# Autodesk Inventor assembly: Top Crossbrace
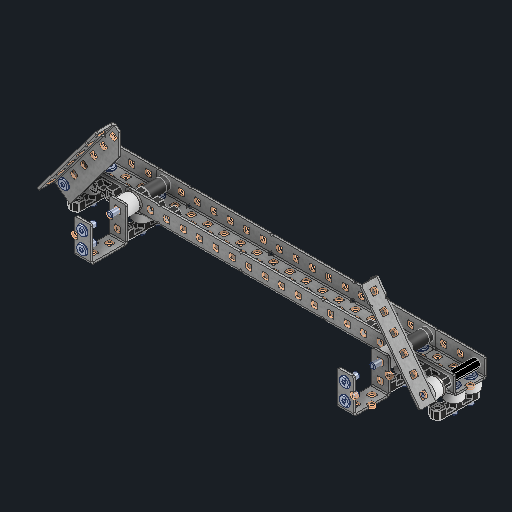
[picture p0: Inventor's stored thumbnail of the model, 512x512]
Saved by Autodesk Inventor 2025 (Build 290162000, 162)
## iProperties
Created: 2024-10-20
Part Number: Top Crossbrace
Document SubType Name: Assembly
Designer: Averey Ku
Author: Averey Ku
## Documents named in this file (26)
- D:\VEX\High Stakes\CAD\V2\Chassis\Structure\Top Crossbrace.iam
- D:\VEX\High Stakes\CAD\ROBOPROS-CAD-Inventor\Structure\C Channel\Aluminum 1x2x1\Alu C 1x2x1x17.ipt
- D:\VEX\High Stakes\CAD\ROBOPROS-CAD-Inventor\Structure\C Channel\Aluminum 2x2x2\Alu C 2x2x2x1.ipt
- D:\VEX\High Stakes\CAD\ROBOPROS-CAD-Inventor\Motion\Spacers\Spacer Nylon .500 OD\NSpacer White .500 OD x .375.ipt
- D:\VEX\High Stakes\CAD\ROBOPROS-CAD-Inventor\Motion\Spacers\Spacer Nylon .500 OD.ipt
- D:\VEX\High Stakes\CAD\ROBOPROS-CAD-Inventor\Motion\Spacers\Washer Steel\SWasher .500 OD x .062500.ipt
- D:\VEX\High Stakes\CAD\ROBOPROS-CAD-Inventor\Motion\Shaft LS\Bearing Flat Low Profile.ipt
- D:\VEX\High Stakes\CAD\ROBOPROS-CAD-Inventor\Motion\Spacers\Washer Steel\SWasher .500 OD x .062500\SWasher .500 OD x .062500.ipt
- D:\VEX\High Stakes\CAD\ROBOPROS-CAD-Inventor\Motion\Spacers\Spacer Nylon .375 OD\NSpacer .375 OD x .125.ipt
- D:\VEX\High Stakes\CAD\ROBOPROS-CAD-Inventor\Motion\Spacers\Spacer Nylon .375 OD.ipt
- D:\VEX\High Stakes\CAD\ROBOPROS-CAD-Inventor\Motion\Spacers\Spacer Nylon .375 OD\NSpacer .375 OD x .500.ipt
- D:\VEX\High Stakes\CAD\ROBOPROS-CAD-Inventor\Structure\Hardware\Screw Steel - Star\SScrew Star Smooth 1.750.ipt
- D:\VEX\High Stakes\CAD\ROBOPROS-CAD-Inventor\Structure\Hardware\Screw Steel - Star.ipt
- D:\VEX\High Stakes\CAD\ROBOPROS-CAD-Inventor\Structure\Hardware\Screw Shoulder Robosource\SScrew Shoulder Smooth .375 x .12.ipt
- D:\VEX\High Stakes\CAD\ROBOPROS-CAD-Inventor\Structure\Hardware\Screw Shoulder Robosource.ipt
- D:\VEX\High Stakes\CAD\ROBOPROS-CAD-Inventor\Motion\Spacers\Spacer Nylon .500 OD\NSpacer White .500 OD x .250.ipt
- D:\VEX\High Stakes\CAD\ROBOPROS-CAD-Inventor\Structure\Hardware\Screw Steel - Star\SScrew Star Smooth .750.ipt
- D:\VEX\High Stakes\CAD\ROBOPROS-CAD-Inventor\Structure\C Channel\Aluminum 1x2x1\Alu C 1x2x1x23.ipt
- D:\VEX\High Stakes\CAD\ROBOPROS-CAD-Inventor\Structure\Standoff\Standoff .875.ipt
- D:\VEX\High Stakes\CAD\ROBOPROS-CAD-Inventor\Structure\Standoff.ipt
- D:\VEX\High Stakes\CAD\ROBOPROS-CAD-Inventor\Structure\C Channel\Aluminum 1x3x1 Half Thick Cut\Alu C Half Thick 1x3x1x6.ipt
- D:\VEX\High Stakes\CAD\ROBOPROS-CAD-Inventor\Structure\Hardware\Screw Steel - Star\SScrew Star Smooth .875.ipt
- D:\VEX\High Stakes\CAD\ROBOPROS-CAD-Inventor\Structure\Hardware\Screw Steel - Star\SScrew Star Smooth .290.ipt
- D:\VEX\High Stakes\CAD\V2\Chassis\Structure\Right\Alu C 2x2x2x1 Right.ipt
- D:\VEX\High Stakes\CAD\V2\Chassis\Structure\Right\Bearing Flat Low Profile Right.ipt
- D:\VEX\High Stakes\CAD\V2\Chassis\Structure\Right\Alu C Half Thick 1x3x1x6 Right.ipt
## Components (54 placed, 19 different names)
1. Alu C 1x2x1x23:1 — Insert:23, Flush:2, Insert:28, Insert:29, Insert:30, Insert:32, Insert:33, Insert:34, Mate:6, Insert:39, Insert:40, Insert:51
2. Alu C 1x2x1x17:1 — Insert:3, Insert:5, Mate:2, Insert:15, Flush:1, Flush:2
3. SScrew Shoulder Smooth .375 x .12:3 — Insert:52
4. Alu C 2x2x2x1:1 — Insert:2, Insert:16, Insert:52
5. NSpacer White .500 OD x .375:1 — Insert:2, Insert:4
6. Bearing Flat Low Profile:1 — Insert:3, Mate:2, Insert:12
7. SWasher .500 OD x .062500:1 — Insert:4, Insert:5, Insert:23
8. NSpacer .375 OD x .125:1 — Insert:11
9. NSpacer .375 OD x .500:2 — Insert:11, Insert:12
10. SScrew Star Smooth 1.750:1 — Insert:15
11. SScrew Shoulder Smooth .375 x .12:1 — Insert:16
12. Alu C Half Thick 1x3x1x6:1 — Insert:33, Insert:36, Insert:38
13. Bearing Flat Low Profile:8 — Insert:34, Mate:6, Insert:37
14. NSpacer White .500 OD x .250:14 — Insert:36
15. SWasher .500 OD x .062500:3 — Insert:37
16. SScrew Star Smooth .875:14 — Insert:38
17. Standoff .875:1 — Insert:39
18. SScrew Star Smooth .290:15 — Insert:40
19. SScrew Shoulder Smooth .375 x .12:4 — Insert:53
20. Alu C 2x2x2x1 Right:1 — Insert:41, Insert:45, Insert:53
21. NSpacer White .500 OD x .375:15 — Insert:41, Insert:42
22. Bearing Flat Low Profile Right:1 — Insert:43
23. SWasher .500 OD x .062500:4 — Insert:42
24. NSpacer .375 OD x .125:3 — Insert:44
25. NSpacer .375 OD x .500:4 — Insert:43, Insert:44
26. SScrew Star Smooth 1.750:16
27. SScrew Shoulder Smooth .375 x .12:2 — Insert:45
28. Alu C Half Thick 1x3x1x6 Right:1 — Insert:48, Insert:50
29. Bearing Flat Low Profile Right:3 — Insert:49
30. NSpacer White .500 OD x .250:18 — Insert:48
31. SWasher .500 OD x .062500:5 — Insert:49
32. SScrew Star Smooth .875:19 — Insert:50
33. Standoff .875:2
34. SScrew Star Smooth .290:20
35. NSpacer White .500 OD x .250:7 — Insert:32
36. NSpacer White .500 OD x .250:6 — Insert:30, Insert:31
37. Bearing Flat Low Profile:4 — Insert:31
38. SScrew Star Smooth .750:7 — Insert:29
39. SScrew Star Smooth .750:6 — Insert:28
40. NSpacer White .500 OD x .250:8
41. NSpacer White .500 OD x .250:9
42. Bearing Flat Low Profile:5
43. SScrew Star Smooth .750:8
44. SScrew Star Smooth .750:9
45. NSpacer White .500 OD x .250:16 — Insert:47, Insert:51
46. NSpacer White .500 OD x .250:17 — Insert:46, Mate:7
47. Bearing Flat Low Profile Right:2 — Insert:46, Insert:47
48. SScrew Star Smooth .750:17
49. SScrew Star Smooth .750:18 — Mate:7
50. NSpacer White .500 OD x .250:19
51. NSpacer White .500 OD x .250:20
52. Bearing Flat Low Profile Right:4
53. SScrew Star Smooth .750:21
54. SScrew Star Smooth .750:22
## Component patterns: Drivebay Attachments Left (2 elements), Drivebay Attachments Right (2 elements)
## Relationships (42: Insert 35, Mate 5, Flush 2)
- [Mate]: Alu C 1x2x1x17:1 ↔ Alu C 2x2x2x1:1
- Insert:2: Alu C 2x2x2x1:1 ↔ NSpacer White .500 OD x .375:1
- Insert:3: Alu C 1x2x1x17:1 ↔ Bearing Flat Low Profile:1
- Insert:4: NSpacer White .500 OD x .375:1 ↔ SWasher .500 OD x .062500:1
- Insert:5: Alu C 1x2x1x17:1 ↔ SWasher .500 OD x .062500:1
- Mate:2: Alu C 1x2x1x17:1 ↔ Bearing Flat Low Profile:1
- Insert:11: NSpacer .375 OD x .125:1 ↔ NSpacer .375 OD x .500:2
- Insert:12 (1.27 mm): Bearing Flat Low Profile:1 ↔ NSpacer .375 OD x .500:2
- Insert:15: Alu C 1x2x1x17:1 ↔ SScrew Star Smooth 1.750:1
- Insert:16: Alu C 2x2x2x1:1 ↔ SScrew Shoulder Smooth .375 x .12:1
- Flush:1 (-107.95 mm): Alu C 1x2x1x17:1
- Insert:23: Alu C 1x2x1x23:1 ↔ SWasher .500 OD x .062500:1
- Flush:2: Alu C 1x2x1x23:1 ↔ Alu C 1x2x1x17:1
- [Mate]: NSpacer White .500 OD x .250:6 ↔ Bearing Flat Low Profile:4
- [Insert] (1.27 mm): NSpacer White .500 OD x .250:7 ↔ Bearing Flat Low Profile:4
- Insert:28: Alu C 1x2x1x23:1 ↔ SScrew Star Smooth .750:6
- Insert:29: Alu C 1x2x1x23:1 ↔ SScrew Star Smooth .750:7
- Insert:30: Alu C 1x2x1x23:1 ↔ NSpacer White .500 OD x .250:6
- Insert:31 (1.27 mm): NSpacer White .500 OD x .250:6 ↔ Bearing Flat Low Profile:4
- Insert:32: Alu C 1x2x1x23:1 ↔ NSpacer White .500 OD x .250:7
- Insert:33 (14.2875 mm): Alu C 1x2x1x23:1 ↔ Alu C Half Thick 1x3x1x6:1
- Insert:34: Alu C 1x2x1x23:1 ↔ Bearing Flat Low Profile:8
- Mate:6: Alu C 1x2x1x23:1 ↔ Bearing Flat Low Profile:8
- Insert:36: Alu C Half Thick 1x3x1x6:1 ↔ NSpacer White .500 OD x .250:14
- Insert:37 (1.27 mm): Bearing Flat Low Profile:8 ↔ SWasher .500 OD x .062500:3
- Insert:38: Alu C Half Thick 1x3x1x6:1 ↔ SScrew Star Smooth .875:14
- Insert:39: Alu C 1x2x1x23:1 ↔ Standoff .875:1
- Insert:40: Alu C 1x2x1x23:1 ↔ SScrew Star Smooth .290:15
- Insert:41: Alu C 2x2x2x1 Right:1 ↔ NSpacer White .500 OD x .375:15
- Insert:42: NSpacer White .500 OD x .375:15 ↔ SWasher .500 OD x .062500:4
- Insert:43 (1.27 mm): Bearing Flat Low Profile Right:1 ↔ NSpacer .375 OD x .500:4
- Insert:44: NSpacer .375 OD x .125:3 ↔ NSpacer .375 OD x .500:4
- Insert:45: Alu C 2x2x2x1 Right:1 ↔ SScrew Shoulder Smooth .375 x .12:2
- Insert:46 (1.27 mm): NSpacer White .500 OD x .250:17 ↔ Bearing Flat Low Profile Right:2
- Insert:47 (1.27 mm): NSpacer White .500 OD x .250:16 ↔ Bearing Flat Low Profile Right:2
- Insert:48: Alu C Half Thick 1x3x1x6 Right:1 ↔ NSpacer White .500 OD x .250:18
- Insert:49 (1.27 mm): Bearing Flat Low Profile Right:3 ↔ SWasher .500 OD x .062500:5
- Insert:50: Alu C Half Thick 1x3x1x6 Right:1 ↔ SScrew Star Smooth .875:19
- Insert:51: Alu C 1x2x1x23:1 ↔ NSpacer White .500 OD x .250:16
- Mate:7: NSpacer White .500 OD x .250:17 ↔ SScrew Star Smooth .750:18
- Insert:52: SScrew Shoulder Smooth .375 x .12:3 ↔ Alu C 2x2x2x1:1
- Insert:53: SScrew Shoulder Smooth .375 x .12:4 ↔ Alu C 2x2x2x1 Right:1
## Named parameters: d46_d43 = 1.27 mm, d47_d31 = 0 mm
